# Autodesk Inventor assembly: endplate_ver2111
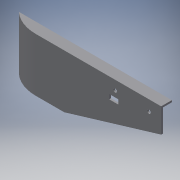
[picture p0: Inventor's stored thumbnail of the model, 180x180]
Saved by Autodesk Inventor 2018.3 (Build 223284000, 284)
## iProperties
Created: 2018-05-29
Part Number: endplate_ver2111
Material: 一般
Document SubType Name: Assembly
Designer: ku_sk
Author: ku_sk
## Documents named in this file (2)
- D:\ku_sk\ドキュメント\Inventor\Aero\KS-15\Fr.wing\parts\endplate\ver.2\endplate_ver2111.iam
- D:\ku_sk\ドキュメント\Inventor\Aero\KS-15\Fr.wing\parts\endplate\ver.2\parts\Part1111.ipt
## Components (1 placed, 1 different names)
1. Part1111:1 — メイト:6, メイト:5, メイト:4
## Relationships (3: Mate 3)
- メイト:6 [Mate]: Part1111:1
- メイト:5 [Mate]: Part1111:1
- メイト:4 [Mate]: Part1111:1
